# Autodesk Inventor assembly: 歯付きベルト伝達
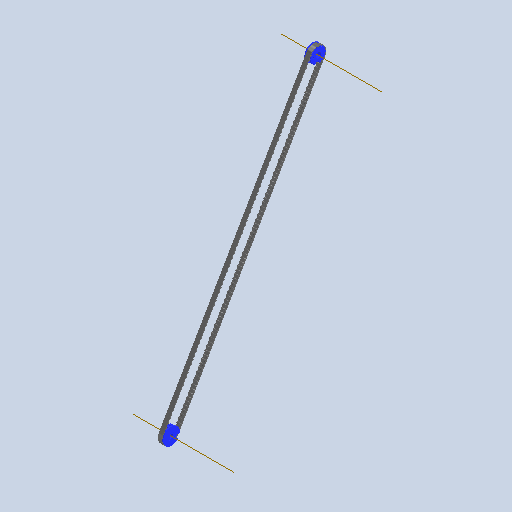
[picture p0: Inventor's stored thumbnail of the model, 512x512]
Saved by Autodesk Inventor 2025.2 (Build 292293000, 293)
## iProperties
ClientObjectVersion: 1
Created: 2025-01-13
Part Number: 歯付きベルト伝達
Document SubType Name: Assembly
Designer: haruy
Author: haruy
## Documents named in this file (4)
- C:\Users\haruy\Documents\ロボコン\NHK2025\cad\nagahisa\belt_liner\000-belt_liner_v2\デザイン アクセラレータ\歯付きベルト伝達2.iam
- C:\Users\haruy\Documents\ロボコン\NHK2025\cad\nagahisa\belt_liner\000-belt_liner_v2\デザイン アクセラレータ\歯付きベルト2.ipt
- C:\Users\haruy\Documents\ロボコン\NHK2025\cad\nagahisa\belt_liner\000-belt_liner_v2\デザイン アクセラレータ\歯付きプーリ11.ipt
- C:\Users\haruy\Documents\ロボコン\NHK2025\cad\nagahisa\belt_liner\000-belt_liner_v2\デザイン アクセラレータ\歯付きプーリ21.ipt
## Components (3 placed, 3 different names)
1. 歯付きベルト:1 — フラッシュ:1, メイト:1, メイト:2, フラッシュ:2, メイト:3, メイト:4
2. 歯付きプーリ1:1 — フラッシュ:1, メイト:1, メイト:2, 回転:1
3. 歯付きプーリ2:1 — フラッシュ:2, メイト:3, 回転:1, メイト:4
## Relationships (7: Mate 4, Flush 2, RelateRotation 1)
- フラッシュ:1 [Flush]: 歯付きベルト:1 ↔ 歯付きプーリ1:1
- メイト:1 [Mate]: 歯付きベルト:1 ↔ 歯付きプーリ1:1
- メイト:2 [Mate]: 歯付きベルト:1 ↔ 歯付きプーリ1:1
- フラッシュ:2 [Flush]: 歯付きベルト:1 ↔ 歯付きプーリ2:1
- メイト:3 [Mate]: 歯付きベルト:1 ↔ 歯付きプーリ2:1
- 回転:1 [RelateRotation] (1 ul): 歯付きプーリ1:1 ↔ 歯付きプーリ2:1
- メイト:4 [Mate]: 歯付きベルト:1 ↔ 歯付きプーリ2:1
